# Autodesk Inventor assembly: camera_mount
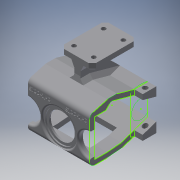
[picture p0: Inventor's stored thumbnail of the model, 180x180]
Saved by Autodesk Inventor 2016 (Build 200138000, 138)
## iProperties
Created: 2016-02-09
Part Number: camera_mount
Document SubType Name: Assembly
Designer: element
Mass: 28.0957 g
Surface Area: 171.888 cm^2
Volume: 28.0957 cm^3
Density: 1 g/cm^3
Author: element
## Documents named in this file (3)
- C:\Users\element\Desktop\technical_drawings\youbot\sensor_mounts\cameras\intel_f200\v3.0\inventor\f200_camera_mount.iam
- C:\Users\element\Desktop\technical_drawings\youbot\sensor_mounts\universal_gripper_sensor_base\v1.0\inventor\universal_gripper_sensor_base.ipt
- C:\Users\element\Desktop\technical_drawings\youbot\sensor_mounts\cameras\intel_f200\v3.0\inventor\f200_camera_head.ipt
## Components (2 placed, 2 different names)
1. universal_gripper_sensor_base:1 — Mate:1, Mate:2, Mate:5
2. f200_camera_head:1 — Mate:1, Mate:2, Mate:5
## Relationships (3: Mate 3)
- Mate:1: universal_gripper_sensor_base:1 ↔ f200_camera_head:1
- Mate:2 (12 mm): universal_gripper_sensor_base:1 ↔ f200_camera_head:1
- Mate:5: universal_gripper_sensor_base:1 ↔ f200_camera_head:1
